# Autodesk Inventor assembly: main
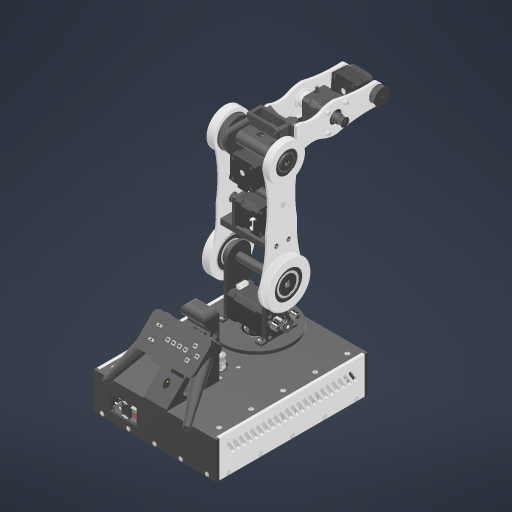
[picture p0: Inventor's stored thumbnail of the model, 512x512]
Saved by Autodesk Inventor 2024.4 (Build 284460000, 460)
## iProperties
Created: 2025-08-25
Part Number: main
Document SubType Name: Assembly
Designer: User
Mass: 2189.26 g
Surface Area: 10547.4 cm^2
Volume: 2189.26 cm^3
Author: User
## Documents named in this file (8)
- C:\Users\Duszy\Desktop\Projekty\Dummy\Dummy_v2\Model\Model\main.iam
- C:\Users\Duszy\Desktop\Projekty\Dummy\Dummy_v2\Model\Model\podstawa\podstawa.iam
- C:\Users\Duszy\Desktop\Projekty\Dummy\Dummy_v2\Model\Model\przegub_1\przegub_0.iam
- C:\Users\Duszy\Desktop\Projekty\Dummy\Dummy_v2\Model\Model\przegub_5\przegub_5.iam
- C:\Users\Duszy\Desktop\Projekty\Dummy\Dummy_v2\Model\Model\przegub_6\przegub_6.iam
- C:\Users\Duszy\Desktop\Projekty\Dummy\Dummy_v2\Model\Model\przegub_4\przegub_4.iam
- C:\Users\Duszy\Desktop\Projekty\Dummy\Dummy_v2\Model\Model\przegub_3\przegub_3.iam
- C:\Users\Duszy\Desktop\Projekty\Dummy\Dummy_v2\Model\Model\przegub_2\przegub_1.iam
## Components (8 placed, 7 different names)
1. podstawa:1 [sub-assembly] — Obrotowe:1
2. przegub_0:1 [sub-assembly] — Obrotowe:1, Sztywne:1, Obrotowe:6
3. przegub_5:1 [sub-assembly] — Obrotowe:4, Obrotowe:5
4. przegub_6:1 [sub-assembly] — Obrotowe:4
5. przegub_4:1 [sub-assembly] — Obrotowe:3, Obrotowe:5
6. przegub_3:1 [sub-assembly] — Obrotowe:2, Obrotowe:3
7. przegub_1:1 [sub-assembly] — Sztywne:1, Obrotowe:2
8. podstawa:2 [sub-assembly] — Obrotowe:6
## Relationships (7: RevoluteJoint 6, WeldJoint 1)
- Obrotowe:1 [RevoluteJoint] (5.25 mm): podstawa:1 ↔ przegub_0:1
- Sztywne:1 [WeldJoint] (-3 mm): przegub_0:1 ↔ przegub_1:1
- Obrotowe:2 [RevoluteJoint] (-0.6 mm): przegub_3:1 ↔ przegub_1:1
- Obrotowe:3 [RevoluteJoint]: przegub_4:1 ↔ przegub_3:1
- Obrotowe:4 [RevoluteJoint]: przegub_5:1 ↔ przegub_6:1
- Obrotowe:5 [RevoluteJoint] (-29 mm): przegub_5:1 ↔ przegub_4:1
- Obrotowe:6 [RevoluteJoint]: przegub_0:1 ↔ podstawa:2
